# Autodesk Inventor assembly: ASY SLM 1662 FDS way 2
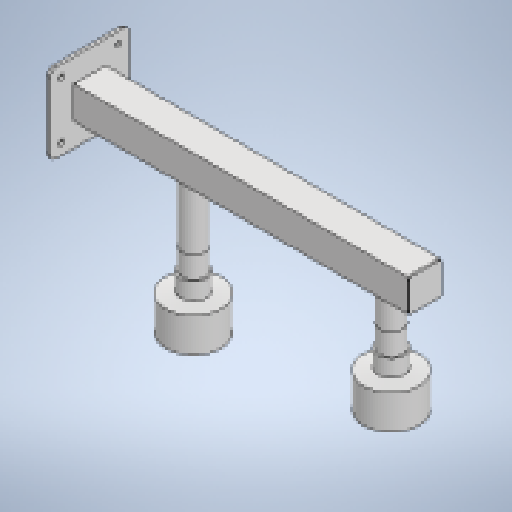
[picture p0: Inventor's stored thumbnail of the model, 512x512]
Saved by Autodesk Inventor 2025.3 (Build 293356030, 356C)
## iProperties
Created: 2025-07-02
Part Number: ASY SLM 1662 FDS way 2
Document SubType Name: Assembly
Designer: admin
Author: user
## Documents named in this file (8)
- C:\Users\admin\Yandex.Disk\home pc\Inventor\SLM Salemal\ASY PNS 1662 FDS way 2.iam
- C:\Users\admin\Yandex.Disk\home pc\Inventor\SLM Salemal\PNS 1662 FDS 1000 way tube 2.ipt
- C:\Users\admin\Yandex.Disk\home pc\Inventor\SLM Salemal\PNS dummy filter element_1600.ipt
- C:\Users\admin\Yandex.Disk\home pc\Inventor\SLM Salemal\PNS dummy pipe nippel_1600.ipt
- C:\Users\admin\Yandex.Disk\home pc\Inventor\SLM Salemal\PNS 1686 FDS 1000 way tube 6.ipt
- C:\Users\admin\Yandex.Disk\home pc\Inventor\SLM Salemal\PNS 1687 FDS 1000 way tube 7.ipt
- C:\Users\admin\Yandex.Disk\home pc\Inventor\SLM Salemal\PNS 1666 FDS 1000 CUP 1.ipt
- C:\Users\admin\Yandex.Disk\home pc\Inventor\SLM Salemal\SLM 1425 FDS Way FLANGE.ipt
## Components (9 placed, 7 different names)
1. PNS 1662 FDS 1000 way tube 2.ipt:1 — Rigid:5, Rigid:8, Rigid:10, Rigid:11
2. PNS 1686 FDS 1000 way tube 6.ipt:1 — Rigid:5, Rigid:4
3. PNS dummy filter element_1600.ipt:2 — Rigid:3
4. PNS dummy pipe nippel_1600.ipt:2 — Rigid:4, Rigid:3
5. PNS 1687 FDS 1000 way tube 7.ipt:1 — Rigid:8, Rigid:7
6. PNS dummy filter element_1600.ipt:3 — Rigid:6
7. PNS dummy pipe nippel_1600.ipt:3 — Rigid:7, Rigid:6
8. PNS 1666 FDS 1000 CUP 1.ipt:1 — Rigid:10
9. SLM 1425 FDS Way FLANGE:1 — Rigid:11
## Relationships (8: WeldJoint 8)
- Rigid:5 [WeldJoint]: PNS 1662 FDS 1000 way tube 2.ipt:1 ↔ PNS 1686 FDS 1000 way tube 6.ipt:1
- Rigid:4 [WeldJoint]: PNS 1686 FDS 1000 way tube 6.ipt:1 ↔ PNS dummy pipe nippel_1600.ipt:2
- Rigid:3 [WeldJoint]: PNS dummy filter element_1600.ipt:2 ↔ PNS dummy pipe nippel_1600.ipt:2
- Rigid:8 [WeldJoint]: PNS 1662 FDS 1000 way tube 2.ipt:1 ↔ PNS 1687 FDS 1000 way tube 7.ipt:1
- Rigid:7 [WeldJoint]: PNS 1687 FDS 1000 way tube 7.ipt:1 ↔ PNS dummy pipe nippel_1600.ipt:3
- Rigid:6 [WeldJoint]: PNS dummy filter element_1600.ipt:3 ↔ PNS dummy pipe nippel_1600.ipt:3
- Rigid:10 [WeldJoint]: PNS 1662 FDS 1000 way tube 2.ipt:1 ↔ PNS 1666 FDS 1000 CUP 1.ipt:1
- Rigid:11 [WeldJoint]: PNS 1662 FDS 1000 way tube 2.ipt:1 ↔ SLM 1425 FDS Way FLANGE:1
